# Autodesk Inventor assembly: PCB
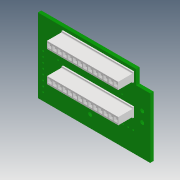
[picture p0: Inventor's stored thumbnail of the model, 180x180]
Saved by Autodesk Inventor 2020 (Build 240168000, 168)
## iProperties
Company: Open CASCADE
Created: 2020-09-27
Part Number: PCB
Description: Open CASCADE Model
Document SubType Name: Assembly
Designer: DELL
Authority: Unknown
Sending System: Open CASCADE 6.8
Preprocessor: Open CASCADE STEP processor 6.8
Title: Open CASCADE Shape Model
Author: Author
## Documents named in this file (3)
- F:\SoftRobot\Model\FlexipodHardware-master\mechanical_model\PCB\PCB.iam
- F:\SoftRobot\Model\FlexipodHardware-master\mechanical_model\PCB\Board.iam
- F:\SoftRobot\Model\FlexipodHardware-master\mechanical_model\PCB\connector.iam
## Components (2 placed, 2 different names)
1. Board_10 [sub-assembly]
2. connector_16 [sub-assembly] — Flush:1
## Relationships (1: Flush 1)
- Flush:1 (-9.374 mm): connector_16
